# Autodesk Inventor assembly: jorge's assembly
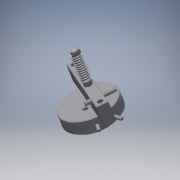
[picture p0: Inventor's stored thumbnail of the model, 180x180]
Saved by Autodesk Inventor 2017.3 (Build 213256000, 256)
## iProperties
Created: 2017-04-26
Part Number: jorge's assembly
Document SubType Name: Assembly
Designer: 167942
Author: 167942
## Documents named in this file (12)
- C:\Users\rbibb\Desktop\8.1\jorge's assembly.iam
- C:\Users\167942.FCBOE\Desktop\Part3.ipt
- C:\Users\167942.FCBOE\Desktop\Part4.ipt
- C:\Users\rbibb\Desktop\8.1\handle pivot pin.ipt
- C:\Users\rbibb\Desktop\8.1\upper die center support.ipt
- C:\Users\rbibb\Desktop\8.1\upper die pressure ring.ipt
- C:\Users\rbibb\Desktop\8.1\upper die center pin.ipt
- C:\Users\167942.FCBOE\Desktop\screw.ipt
- C:\Users\rbibb\Desktop\8.1\Large Snap Ring.ipt
- C:\Users\rbibb\Desktop\8.1\Upper Die Spring (1).ipt
- C:\Users\rbibb\Desktop\8.1\upper die outter ring.ipt
- C:\Users\rbibb\Desktop\8.1\upper die center.ipt
## Components (11 placed, 11 different names)
1. Part3:1 — Rotational:4
2. Part4:1 — Rotational:5, Rotational:6
3. handle pivot pin:1 — Cylindrical:1
4. upper die center support:1 — Cylindrical:1, Rigid:1, Rotational:3
5. upper die pressure ring:1 — Rotational:3, Rotational:4, Rotational:5, Rotational:9, Rotational:10
6. upper die center pin:1 — Rigid:1, Rotational:7
7. screw:1 — Rotational:6
8. Large Snap Ring:1 — Rotational:7, Rotational:8
9. Upper Die Spring (1):1 — Rotational:8
10. upper die outter ring:1 — Rotational:9
11. upper die center:1 — Rotational:10
## Relationships (10: RevoluteJoint 8, CylindricalJoint 1, WeldJoint 1)
- Cylindrical:1: handle pivot pin:1 ↔ upper die center support:1
- Rigid:1 [WeldJoint]: upper die center support:1 ↔ upper die center pin:1
- Rotational:3 [RevoluteJoint]: upper die center support:1 ↔ upper die pressure ring:1
- Rotational:4 [RevoluteJoint]: Part3:1 ↔ upper die pressure ring:1
- Rotational:5 [RevoluteJoint]: Part4:1 ↔ upper die pressure ring:1
- Rotational:6 [RevoluteJoint]: Part4:1 ↔ screw:1
- Rotational:7 [RevoluteJoint]: upper die center pin:1 ↔ Large Snap Ring:1
- Rotational:8 [RevoluteJoint]: Large Snap Ring:1 ↔ Upper Die Spring (1):1
- Rotational:9 [RevoluteJoint]: upper die pressure ring:1 ↔ upper die outter ring:1
- Rotational:10 [RevoluteJoint]: upper die pressure ring:1 ↔ upper die center:1
